# Autodesk Inventor assembly: Assembly2
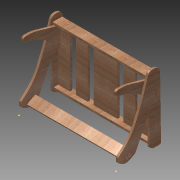
[picture p0: Inventor's stored thumbnail of the model, 180x180]
Saved by Autodesk Inventor 2015 (Build 190159000, 159)
## iProperties
Created: 2016-02-10
Part Number: Assembly2
Document SubType Name: Assembly
Designer: iberopuebla
Author: iberopuebla
## Documents named in this file (8)
- C:\Users\iberopuebla.IBERO\Documents\Futón bien\Assembly2.iam
- C:\Users\iberopuebla.IBERO\Documents\Futón bien\Pata con lado.ipt
- C:\Users\iberopuebla.IBERO\Documents\Futón bien\Pata.ipt
- C:\Users\iberopuebla.IBERO\Documents\Futón bien\Viga delantera.ipt
- C:\Users\iberopuebla.IBERO\Documents\Futón bien\viga diagonal.ipt
- C:\Users\iberopuebla.IBERO\Documents\Futón bien\Viga trasera.ipt
- C:\Users\iberopuebla.IBERO\Documents\Futón bien\laterales.ipt
- C:\Users\iberopuebla.IBERO\Documents\Futón bien\vigas.ipt
## Components (13 placed, 7 different names)
1. Pata con lado:1 — Mate:4, Mate:5, Mate:6, Mate:7, Mate:10, Mate:11
2. Pata:1 — Mate:7, Mate:32, Mate:33
3. Viga delantera:1 — Mate:4, Mate:5, Mate:6, Mate:30, Mate:31, Mate:34, Mate:35
4. viga diagonal:1
5. Viga trasera:1 — Mate:10, Mate:11, Mate:19, Mate:20, Mate:21, Mate:22, Mate:23, Mate:24, Mate:25, Mate:26, Mate:27
6. Pata:2 — Mate:29
7. laterales:1 — Mate:29
8. laterales:2 — Mate:30, Mate:31, Mate:32, Mate:33
9. vigas:1 — Mate:22, Mate:23
10. vigas:2 — Mate:19, Mate:20, Mate:21
11. vigas:3 — Mate:24, Mate:25
12. vigas:4 — Mate:26, Mate:27
13. Pata con lado:2 — Mate:34, Mate:35
## Relationships (22: Mate 22)
- Mate:4: Pata con lado:1 ↔ Viga delantera:1
- Mate:5: Pata con lado:1 ↔ Viga delantera:1
- Mate:6: Pata con lado:1 ↔ Viga delantera:1
- Mate:7: Pata con lado:1 ↔ Pata:1
- Mate:10: Pata con lado:1 ↔ Viga trasera:1
- Mate:11: Pata con lado:1 ↔ Viga trasera:1
- Mate:19: Viga trasera:1 ↔ vigas:2
- Mate:20: Viga trasera:1 ↔ vigas:2
- Mate:21: Viga trasera:1 ↔ vigas:2
- Mate:22: Viga trasera:1 ↔ vigas:1
- Mate:23: Viga trasera:1 ↔ vigas:1
- Mate:24: Viga trasera:1 ↔ vigas:3
- Mate:25: Viga trasera:1 ↔ vigas:3
- Mate:26: Viga trasera:1 ↔ vigas:4
- Mate:27: Viga trasera:1 ↔ vigas:4
- Mate:29: Pata:2 ↔ laterales:1
- Mate:30: Viga delantera:1 ↔ laterales:2
- Mate:31: Viga delantera:1 ↔ laterales:2
- Mate:32: Pata:1 ↔ laterales:2
- Mate:33: Pata:1 ↔ laterales:2
- Mate:34: Viga delantera:1 ↔ Pata con lado:2
- Mate:35: Viga delantera:1 ↔ Pata con lado:2
